# Autodesk Inventor assembly: КВ33.044.300 -  Сборка мотора Makeblock с крепление
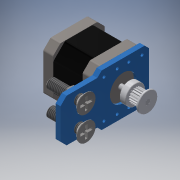
[picture p0: Inventor's stored thumbnail of the model, 180x180]
Saved by Autodesk Inventor 2019 (Build 230136000, 136)
## iProperties
Created: 2019-07-17
Part Number: КВ33.044.300 -  Сборка мотора Makeblock с крепление
Material: Типовые
Document SubType Name: Assembly
Designer: Петров Иван
Author: Петров Иван
## Documents named in this file (6)
- E:\IVAN\Kvantoriada2019\optimal_gripper\hardware\КВ33.044.300 -  Сборка мотора Makeblock с крепление.iam
- E:\IVAN\Kvantoriada2019\optimal_gripper\hardware\КВ33.044.301 - Деражатель мотора.ipt
- E:\IVAN\Kvantoriada2019\optimal_gripper\hardware\Стандартные изделия\Шаговый двигатель Makeblock.ipt
- E:\IVAN\Kvantoriada2019\optimal_gripper\hardware\Стандартные изделия\шкив Makeblock.ipt
- E:\IVAN\Kvantoriada2019\optimal_gripper\hardware\Стандартные изделия\Винт М8х25 с потайной головкой.ipt
- C:\Users\Петров Иван\Documents\Inventor\Content Center Files\R2019\ru-RU\AS 1112 (4)\AS 1112 - M6(2).ipt
## Components (7 placed, 5 different names)
1. КВ33.044.301 - Деражатель мотора:1 — Совмещение:1, Совмещение:2, Совмещение:3, Совмещение:5, Совмещение:6, Заподлицо:1, Совмещение:7, Заподлицо:2, Вставка:1, Вставка:2
2. Шаговый двигатель Makeblock:1 — Совмещение:1, Совмещение:2, Совмещение:3, Совмещение:4
3. шкив Makeblock:1 — Совмещение:4, Совмещение:5
4. Винт М8х25 с потайной головкой:1 — Совмещение:6, Заподлицо:1
5. Винт М8х25 с потайной головкой:2 — Совмещение:7, Заподлицо:2
6. AS 1112 (4) - метрическая M6:1 — Вставка:1
7. AS 1112 (4) - метрическая M6:2 — Вставка:2
## Relationships (11: Mate 7, Flush 2, Insert 2)
- Совмещение:1 [Mate]: КВ33.044.301 - Деражатель мотора:1 ↔ Шаговый двигатель Makeblock:1
- Совмещение:2 [Mate]: КВ33.044.301 - Деражатель мотора:1 ↔ Шаговый двигатель Makeblock:1
- Совмещение:3 [Mate]: КВ33.044.301 - Деражатель мотора:1 ↔ Шаговый двигатель Makeblock:1
- Совмещение:4 [Mate]: Шаговый двигатель Makeblock:1 ↔ шкив Makeblock:1
- Совмещение:5 [Mate] (5 mm): КВ33.044.301 - Деражатель мотора:1 ↔ шкив Makeblock:1
- Совмещение:6 [Mate]: КВ33.044.301 - Деражатель мотора:1 ↔ Винт М8х25 с потайной головкой:1
- Заподлицо:1 [Flush] (-6 mm): КВ33.044.301 - Деражатель мотора:1 ↔ Винт М8х25 с потайной головкой:1
- Совмещение:7 [Mate]: КВ33.044.301 - Деражатель мотора:1 ↔ Винт М8х25 с потайной головкой:2
- Заподлицо:2 [Flush] (-6 mm): КВ33.044.301 - Деражатель мотора:1 ↔ Винт М8х25 с потайной головкой:2
- Вставка:1 [Insert]: КВ33.044.301 - Деражатель мотора:1 ↔ AS 1112 (4) - метрическая M6:1
- Вставка:2 [Insert]: КВ33.044.301 - Деражатель мотора:1 ↔ AS 1112 (4) - метрическая M6:2
